# Autodesk Inventor assembly: complete
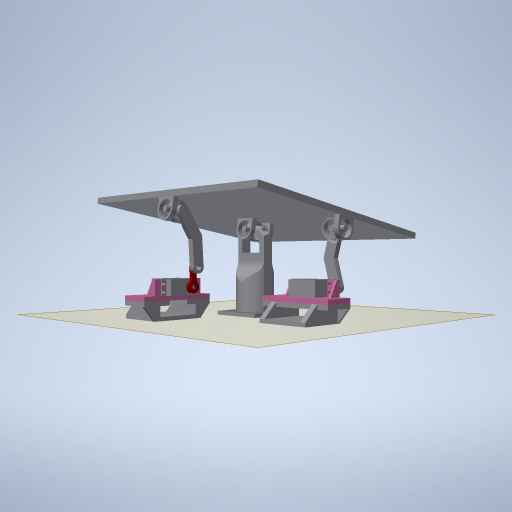
[picture p0: Inventor's stored thumbnail of the model, 512x512]
Saved by Autodesk Inventor 2024 (Build 280153000, 153)
## iProperties
Created: 2024-04-03
Part Number: complete
Document SubType Name: Assembly
Designer: compu
Author: compu
## Documents named in this file (11)
- C:\Users\compu\Documents\1Juan\1Facultad\9 Semestre\E1225 Taller de Sistemas Digitales\Parts\complete.iam
- C:\Users\compu\Documents\1Juan\1Facultad\9 Semestre\E1225 Taller de Sistemas Digitales\Parts\tabla40.ipt
- C:\Users\compu\Documents\1Juan\1Facultad\9 Semestre\E1225 Taller de Sistemas Digitales\Parts\center piece\anillo central.ipt
- C:\Users\compu\Documents\1Juan\1Facultad\9 Semestre\E1225 Taller de Sistemas Digitales\Parts\center piece\laterales.ipt
- C:\Users\compu\Documents\1Juan\1Facultad\9 Semestre\E1225 Taller de Sistemas Digitales\Parts\borde dos piezas\borde libre.ipt
- C:\Users\compu\Documents\1Juan\1Facultad\9 Semestre\E1225 Taller de Sistemas Digitales\Parts\borde dos piezas\side arm.ipt
- C:\Users\compu\Documents\1Juan\1Facultad\9 Semestre\E1225 Taller de Sistemas Digitales\Parts\25T M3.ipt
- C:\Users\compu\Documents\1Juan\1Facultad\9 Semestre\E1225 Taller de Sistemas Digitales\Componentes\Servos\MG996R.ipt
- C:\Users\compu\Documents\1Juan\1Facultad\9 Semestre\E1225 Taller de Sistemas Digitales\Parts\borde dos piezas\pilar central.ipt
- C:\Users\compu\Documents\1Juan\1Facultad\9 Semestre\E1225 Taller de Sistemas Digitales\Parts\soporte servo\soporte sup.ipt
- C:\Users\compu\Documents\1Juan\1Facultad\9 Semestre\E1225 Taller de Sistemas Digitales\Parts\soporte servo\soporte infe.ipt
## Components (19 placed, 10 different names)
1. anillo central:1 — Mate:1, Flush:1, Mate:2, Flush:2, Mate:3, Flush:3, Mate:28, Mate:56, Mate:68
2. laterales:1 — Mate:2, Flush:2, Mate:5, Mate:11, Mate:13, Mate:16, Mate:18, Mate:21
3. laterales:2 — Mate:3, Flush:3, Mate:4, Mate:10, Mate:15, Mate:17
4. tabla40:1 — Mate:4, Mate:5, Mate:6, Mate:7, Mate:23, Mate:24, Mate:25, Flush:4, Mate:30, Flush:5, Mate:33
5. laterales:3 — Mate:32, Flush:5, Mate:33, Mate:35, Flush:7
6. laterales:4 — Mate:29, Flush:4, Mate:30, Mate:34, Flush:6
7. borde libre:1 — Mate:34, Flush:6, Flush:9, Mate:37, Mate:54, Mate:68
8. borde libre:2 — Mate:35, Flush:7, Flush:8, Mate:38, Mate:39
9. side arm:1 — Mate:38, Mate:39, Mate:42, Mate:43
10. side arm:2 — Mate:37, Mate:40, Mate:41, Mate:54
11. 25T M3:1 — Mate:42, Mate:43, Mate:44, Mate:45, Angle:4
12. 25T M3:2 — Mate:40, Mate:41, Mate:47, Mate:48, Angle:3
13. MG996R:1 — Mate:44, Mate:45, Mate:53, Flush:12, Angle:4, Mate:58, Mate:59, Mate:60
14. MG996R:2 — Mate:47, Mate:48, Mate:50, Mate:51, Angle:3, Mate:61, Mate:62, Mate:63
15. pilar central:1 — Mate:55, Mate:56, Mate:57
16. soporte sup:1 — Mate:58, Mate:59, Mate:60, Flush:14, Mate:64, Flush:15
17. soporte sup:2 — Mate:61, Mate:62, Mate:63, Flush:16, Mate:66, Flush:17
18. soporte infe:1 — Flush:14, Mate:64, Flush:15, Mate:65
19. soporte infe:2 — Flush:16, Mate:66, Flush:17, Mate:67
## Relationships (82: Mate 64, Flush 16, Angle 2)
- Mate:1: anillo central:1
- Flush:1 (4 mm): anillo central:1
- Mate:2: anillo central:1 ↔ laterales:1
- Flush:2: anillo central:1 ↔ laterales:1
- Mate:3: anillo central:1 ↔ laterales:2
- Flush:3: anillo central:1 ↔ laterales:2
- Mate:4: laterales:2 ↔ tabla40:1
- Mate:5: laterales:1 ↔ tabla40:1
- Mate:6: tabla40:1
- Mate:7: tabla40:1
- Mate:8
- Mate:9
- Mate:10: laterales:2
- Mate:11: laterales:1
- Mate:12
- Mate:13: laterales:1
- Mate:14
- Mate:15: laterales:2
- Mate:16: laterales:1
- Mate:17: laterales:2
- Mate:18: laterales:1
- Mate:19
- Mate:20
- Mate:21: laterales:1
- Mate:22
- Mate:23: tabla40:1
- Mate:24: tabla40:1
- Mate:25: tabla40:1
- Mate:26
- Mate:27
- Mate:28: anillo central:1
- Mate:29: laterales:4
- Flush:4: tabla40:1 ↔ laterales:4
- Mate:30: tabla40:1 ↔ laterales:4
- Mate:31
- Mate:32: laterales:3
- Flush:5: tabla40:1 ↔ laterales:3
- Mate:33: tabla40:1 ↔ laterales:3
- Mate:34: laterales:4 ↔ borde libre:1
- Flush:6: laterales:4 ↔ borde libre:1
- Mate:35: laterales:3 ↔ borde libre:2
- Flush:7: laterales:3 ↔ borde libre:2
- Flush:8 (4 mm): borde libre:2
- Flush:9 (4 mm): borde libre:1
- Mate:37: borde libre:1 ↔ side arm:2
- Mate:38: borde libre:2 ↔ side arm:1
- Mate:39: borde libre:2 ↔ side arm:1
- Mate:40: side arm:2 ↔ 25T M3:2
- Mate:41 (0.5 mm): side arm:2 ↔ 25T M3:2
- Mate:42: side arm:1 ↔ 25T M3:1
- Mate:43 (0.5 mm): side arm:1 ↔ 25T M3:1
- Flush:11 (-80 mm)
- Mate:44: 25T M3:1 ↔ MG996R:1
- Mate:45: 25T M3:1 ↔ MG996R:1
- Mate:47: 25T M3:2 ↔ MG996R:2
- Mate:48: 25T M3:2 ↔ MG996R:2
- Mate:50: MG996R:2
- Mate:51 (90.13 mm): MG996R:2
- Mate:53: MG996R:1
- Flush:12 (-90.13 mm): MG996R:1
- Flush:13 (-30 mm)
- Angle:3 (90 deg): 25T M3:2 ↔ MG996R:2
- Angle:4 (0 deg): 25T M3:1 ↔ MG996R:1
- Mate:54: borde libre:1 ↔ side arm:2
- Mate:55: pilar central:1
- Mate:56 (2 mm): anillo central:1 ↔ pilar central:1
- Mate:57: pilar central:1
- Mate:58: MG996R:1 ↔ soporte sup:1
- Mate:59: MG996R:1 ↔ soporte sup:1
- Mate:60: MG996R:1 ↔ soporte sup:1
- Mate:61: MG996R:2 ↔ soporte sup:2
- Mate:62: MG996R:2 ↔ soporte sup:2
- Mate:63: MG996R:2 ↔ soporte sup:2
- Flush:14: soporte sup:1 ↔ soporte infe:1
- Mate:64: soporte sup:1 ↔ soporte infe:1
- Flush:15: soporte sup:1 ↔ soporte infe:1
- Mate:65: soporte infe:1
- Flush:16: soporte sup:2 ↔ soporte infe:2
- Mate:66: soporte sup:2 ↔ soporte infe:2
- Flush:17: soporte sup:2 ↔ soporte infe:2
- Mate:67: soporte infe:2
- Mate:68: anillo central:1 ↔ borde libre:1
## Named parameters: Finish1_Area = 1896
note: some values were not read from the file. Shown as the stored number, unit unknown: "Finish1_Area".
